# Autodesk Inventor assembly: 4 Omni, Circle_MIR
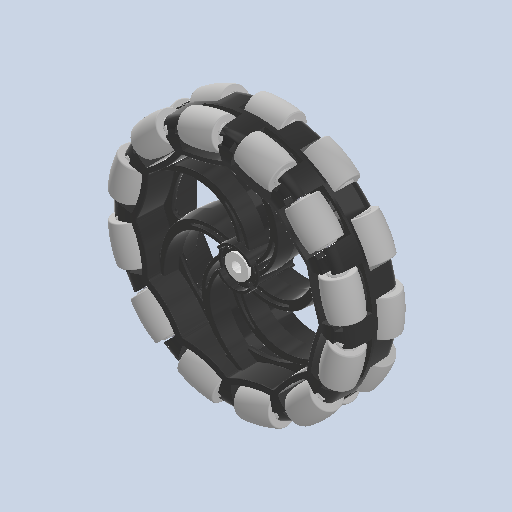
[picture p0: Inventor's stored thumbnail of the model, 512x512]
Saved by Autodesk Inventor 2024 (Build 280153000, 153)
## iProperties
Created: 2022-08-02
Part Number: 4 Omni, Circle_MIR
Document SubType Name: Assembly
Designer: ismae
Author: ylu12
## Documents named in this file (3)
- C:\Users\ismae\Desktop\VEX\CAD 2023\VEX-CAD-Inventor\Motion\Wheels\Omni Wheel\4 Omni, Circle_MIR.iam
- C:\Users\ismae\Desktop\VEX\CAD 2023\VEX-CAD-Inventor\Motion\Wheels\Reference Files\4 Omni_MIR.ipt
- C:\Users\ismae\Desktop\VEX\CAD 2023\VEX-CAD-Inventor\Motion\Insert Circle_MIR1.ipt
## Components (3 placed, 2 different names)
1. 4 Omni_MIR:1 — Nivelación:8, Coincidencia:16, Coincidencia:15
2. Insert Circle_MIR1:1 — Ángulo:2, Coincidencia:20, Nivelación:13, Nivelación:12, Nivelación:14
3. Insert Circle_MIR1:2 — Nivelación:13, Nivelación:12, Coincidencia:19
## Relationships (9: Flush 4, Mate 4, Angle 1)
- Nivelación:8 [Flush]: 4 Omni_MIR:1
- Coincidencia:16 [Mate]: 4 Omni_MIR:1
- Coincidencia:15 [Mate]: 4 Omni_MIR:1
- Ángulo:2 [Angle] (0 deg): Insert Circle_MIR1:1
- Coincidencia:20 [Mate]: Insert Circle_MIR1:1
- Nivelación:13 [Flush]: Insert Circle_MIR1:1 ↔ Insert Circle_MIR1:2
- Nivelación:12 [Flush]: Insert Circle_MIR1:1 ↔ Insert Circle_MIR1:2
- Nivelación:14 [Mate] (7.0104 mm): Insert Circle_MIR1:1
- Coincidencia:19 [Flush] (7.0104 mm): Insert Circle_MIR1:2
